# Autodesk Inventor assembly: Odom Pod
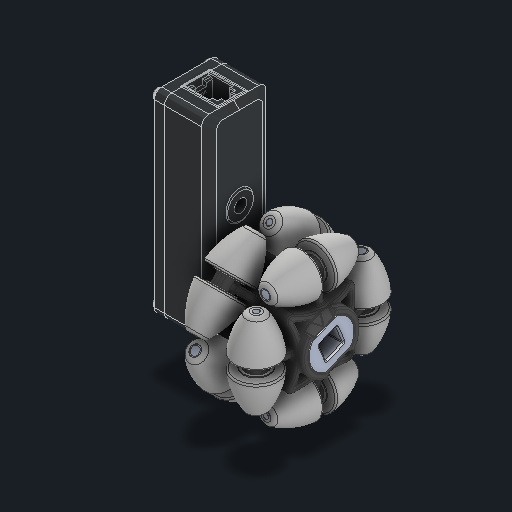
[picture p0: Inventor's stored thumbnail of the model, 512x512]
Saved by Autodesk Inventor 2025.1 (Build 291241000, 241)
## iProperties
Created: 2025-01-13
Part Number: Odom Pod
Document SubType Name: Assembly
Designer: avere
Author: avere
## Documents named in this file (3)
- C:\Users\avere\VEX\High Stakes\CAD\V4\Chassis\Odom Pod.iam
- C:\Users\avere\VEX\High Stakes\CAD\ROBOPROS-CAD-Inventor\Electronics\Sensors\V5 Rotation Sensor.ipt
- C:\Users\avere\VEX\High Stakes\CAD\ROBOPROS-CAD-Inventor\Motion\Wheels\Omni Wheel\2.00 Omni AS, No Insert.ipt
## Components (3 placed, 2 different names)
1. V5 Rotation Sensor:1 — Insert:2
2. 2.00 Omni AS, No Insert:1 — Insert:1, Flush:1
3. 2.00 Omni AS, No Insert:2 — Insert:1, Flush:1, Insert:2
## Relationships (3: Insert 2, Flush 1)
- Insert:1: 2.00 Omni AS, No Insert:1 ↔ 2.00 Omni AS, No Insert:2
- Flush:1: 2.00 Omni AS, No Insert:1 ↔ 2.00 Omni AS, No Insert:2
- Insert:2: V5 Rotation Sensor:1 ↔ 2.00 Omni AS, No Insert:2
